# Autodesk Inventor assembly: omniAssembly
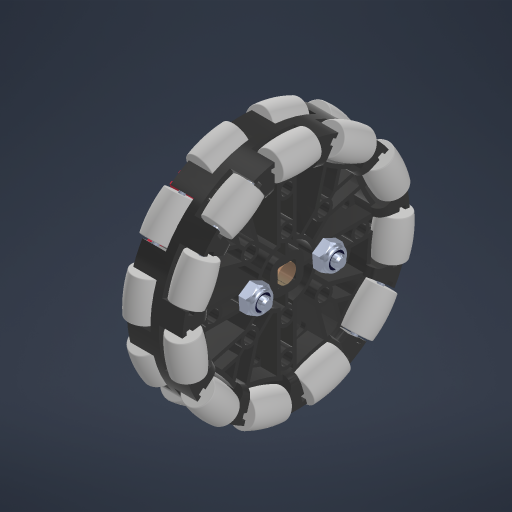
[picture p0: Inventor's stored thumbnail of the model, 512x512]
Saved by Autodesk Inventor 2023.4 (Build 274418000, 418)
## iProperties
Created: 2024-03-08
Part Number: omniAssembly
Document SubType Name: Assembly
Designer: Meer
Author: Meer
## Documents named in this file (9)
- C:\Users\Meer\OneDrive\Documents\worlds bot possibly\omniAssembly.iam
- C:\Users\Meer\OneDrive\Documents\GitHub\2024-599Z\Cad\Library\VEX-CAD-Inventor-1.4.0\Motion\Wheels\Omni Wheel\3.25 Omni AS, No Insert.iam
- C:\Users\Meer\OneDrive\Documents\GitHub\2024-599Z\Cad\Library\VEX-CAD-Inventor-1.4.0\Motion\Wheels\Omni Wheel.iam
- C:\Users\Meer\OneDrive\Documents\worlds bot possibly\42tHalfcut.iam
- C:\Users\Meer\OneDrive\Documents\GitHub\2024-599Z\Cad\Library\VEX-CAD-Inventor-1.4.0\Structure\Hardware\Nut Thin Nylock.ipt
- C:\Users\Meer\OneDrive\Documents\GitHub\2024-599Z\Cad\Library\VEX-CAD-Inventor-1.4.0\Structure\Hardware\Screw Steel - Star\SScrew Star Smooth 1.250.ipt
- C:\Users\Meer\OneDrive\Documents\GitHub\2024-599Z\Cad\Library\VEX-CAD-Inventor-1.4.0\Structure\Hardware\Screw Steel - Star.ipt
- C:\Users\Meer\OneDrive\Documents\GitHub\2024-599Z\Cad\Library\VEX-CAD-Inventor-1.4.0\Motion\Spacers\Spacer Nylon .375 OD\NSpacer .375 OD x .250.ipt
- C:\Users\Meer\OneDrive\Documents\GitHub\2024-599Z\Cad\Library\VEX-CAD-Inventor-1.4.0\Motion\Spacers\Spacer Nylon .375 OD.ipt
## Components (8 placed, 5 different names)
1. 3.25 Omni AS, No Insert:1 [sub-assembly]
2. 42tHalfcut:1 [sub-assembly]
3. Nut Thin Nylock:1
4. SScrew Star Smooth 1.250:1
5. NSpacer .375 OD x .250:1
6. SScrew Star Smooth 1.250:2
7. NSpacer .375 OD x .250:2
8. Nut Thin Nylock:2
## Relationships (9: Insert 9)
- [Insert]: 3.25 Omni AS, No Insert:1 ↔ 42tHalfcut:1
- [Insert]: 42tHalfcut:1 ↔ SScrew Star Smooth 1.250:1
- [Insert]: 3.25 Omni AS, No Insert:1 ↔ NSpacer .375 OD x .250:1
- [Insert]: 42tHalfcut:1 ↔ NSpacer .375 OD x .250:1
- [Insert]: 42tHalfcut:1 ↔ SScrew Star Smooth 1.250:2
- [Insert]: 3.25 Omni AS, No Insert:1 ↔ NSpacer .375 OD x .250:2
- [Insert]: 42tHalfcut:1 ↔ NSpacer .375 OD x .250:2
- [Insert]: 3.25 Omni AS, No Insert:1 ↔ Nut Thin Nylock:1
- [Insert]: 3.25 Omni AS, No Insert:1 ↔ Nut Thin Nylock:2
